# Autodesk Inventor assembly: ATP16XL025-A-P8
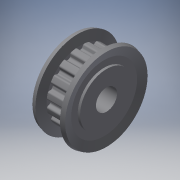
[picture p0: Inventor's stored thumbnail of the model, 180x180]
Saved by Autodesk Inventor 2019 (Build 230136000, 136)
## iProperties
Category: PARTsolutions
Company: MISUMI
Created: 2024-03-16
Part Number: ATP16XL025-A-P8
Catalog Web Link: www.cadenas.de
Description: ATP__XL025, ATP__XL031, ATP__ XL037, ATP__XL050, BTP__XL025, BTP__XL031, BTP__XL037, BTP__XL050, KTP__XL025, KTP__XL031, KTP__ XL037, KTP__XL050, NTP__XL025, NTP__XL031, NTP__ XL037, NTP__XL050, MTP__XL025, MTP__ XL037, MTP__XL050, MTPB__XL025, MTPB__ XL037, MTPB__XL050, MTPP__XL025, MTPP__ XL037, MTPP__XL050, STP__XL025, STP__XL031, STP__ XL037, STP__XL050, KATP__XL025, KATP__XL031, KATP__ XL037, KATP__XL050, KKTP__XL025, KKTP__XL031, KKTP__ XL037, KKTP__XL050-Timing Pulleys XL Type
Vendor: MISUMI
Document SubType Name: Assembly
Designer: psAdmin
Manufacturer: MISUMI
Mass: 5.87054 g
Surface Area: 39.0315 cm^2
Volume: 5.87054 cm^3
Density: 1 g/cm^3
Title: ATP16XL025-A-P8
Author: Cadenas PARTsolutions
Comments: Timing Pulleys XL Type
PSOL_IDENT_0: {$CADENAS_DATA/23d-libs/misumi/metric/51_timing_pulleys/mtp_xl_asmtab.prj},892 {VTYP=3D},{STYP=ASSTA
PSOL_IDENT_1: B},{NB=ATP16XL025-A-P8},{LINA=ATP16XL025-A-P8},{NN=ATP__XL025, ATP__XL031, ATP__ XL037, ATP__XL050,
PSOL_IDENT_2: BTP__XL025, BTP__XL031, BTP__XL037, BTP__XL050, KTP__XL025, KTP__XL031, KTP__ XL037, KTP__XL050, NTP
PSOL_IDENT_3: __XL025, NTP__XL031, NTP__ XL037, NTP__XL050, MTP__XL025, MTP__ XL037, MTP__XL050, MTPB__XL025, MTPB
PSOL_IDENT_4: __ XL037, MTPB__XL050, MTPP__XL025, MTPP__ XL037, MTPP__XL050, STP__XL025, STP__XL031, STP__ XL037,
PSOL_IDENT_5: STP__XL050, KATP__XL025, KATP__XL031, KATP__ XL037, KATP__XL050, KKTP__XL025, KKTP__XL031, KKTP__ XL
PSOL_IDENT_6: 037, KKTP__XL050},{DATE=06.01.2023 09:05:48},{GEOMDATE=06.01.2023 09:05:40},{VERSION=},{LINEID=30},{
PSOL_IDENT_7: WBVAR=MATP,ST,TNW,PS,SBS,DD,Z,J,Q,R,S,T,ALT1,ALT2,M,QSC,QFC,QTC,ALT3,K,KSC,KFC,KTC,ALT4,ZM,ZSC,ZFC,Z
PSOL_IDENT_8: TC,ALT5,ALT6,ALT7,FC,ALT8,SRG,ALT9,BTC,TL,ALT10,TPC,ALT11,BC,ALT12,SLH,ALT13,BN},{WBNUMERIC=DD,Z,J,Q
PSOL_IDENT_9: ,R,S,T,QSC,QFC,QTC,K,KSC,KFC,KTC,ZSC,ZFC,ZTC,FC,SRG,BTC,TL,BC,SLH,BN}  {NB=ATP16XL025-A-P8},{LINA=AT
PSOL_IDENT_10: P16XL025-A-P8},{KT=DUMMY},{PN=ATP16XL025-A-P8},{TYPE=ATP},{MATP=A2017},{MATPALG= 'A2017','Aluminum A
PSOL_IDENT_11: lloy 2000 series','S45C','1045 Carbon Steel Equivalent','SUS304','SUS304', 'A6000', '6000 Series Alu
PSOL_IDENT_12: minum Alloy' },{ST=CA},{STALG= 'CA','Clear Anodize','BA','Black Anodize','HAT','Hard Clear Anodize','
PSOL_IDENT_13: ENP','Electroless Nickel Plating' },{NT=16},{TNW=XL025},{TNWALG= 'XL025','XL031','XL037','XL050' },{
PSOL_IDENT_14: BW=6.4mm (1/4inch)},{PS=A},{PSALG= 'A','B' },{SBS=P},{SBSALG= 'H','Round Hole','P','Round Hole + Tap'
PSOL_IDENT_15: ,'N','New JIS Keywayed Bore + Tap (Standard)','NK','New JIS Keywayed Bore + Tap (width 4.0mm, height
PSOL_IDENT_16: 1.8mm)','C','Old JIS Keywayed Bore + Tap','V','Stepped Hole','Y','Both Ends Stepped Hole','WB','Dou
PSOL_IDENT_17: ble Stepped Hole' },{DD=8.00},{DDALG=[5:6/1],6.35,[7:12/1],12.7,[13:13/1]},{DDHA=[5:6/1],6.35,[7:12/
PSOL_IDENT_18: 1],12.7,[13:16/1]},{DDPA=[5:6/1],6.35,[7:12/1],12.7,[13:13/1]},{DDNA=[8:8/1],[10:13/1]},{DDNK=[10:10
PSOL_IDENT_19: /1]},{DDCA=[10,12]},{DDVA=[5:6/1],6.35,[7:12/1],12.7,[13:14/1]},{DDY=[5:14/1]},{DDWB=[5:12/1]},{DDHB=
PSOL_IDENT_20: },{DDPB=},{DDNB=},{DDCB=},{DDVFB=},{Z=0},{ZALG=[0]},{ZMIN=10.000},{ZAMAX=16.000},{ZBMAX=0.000},{DDZ=
PSOL_IDENT_21: 8.000},{J=0.0},{JALG=[0]},{JMIN=2.000},{JMAX=10.500},{JPN=},{Q=0},{QALG=[0]},{QRMIN=10.000},{QRMAX=1
PSOL_IDENT_22: 6},{WBQMIN=12.000},{R=0},{RALG=[0]},{WBRMAX=-2.000},{S=0.0},{SALG=[0]},{SMAX=6.5},{T=0.0},{TALG=[0]}
PSOL_IDENT_23: ,{TMAX=8},{SBSPN=-P8},{A=7.5},{W=12.5},{L=0},{PD=25.87},{OD=25.36},{D=0},{DALG=17.000},{DE=20},{F=32
PSOL_IDENT_24: },{E=20},{TT=1.6},{BBK=0.000},{TTK=0.0},{ALT1=},{ALT1ALG= '','w/o KC90 (Set Screw Angle)','KC90','wi
PSOL_IDENT_25: th KC90 (Set Screw Angle)' },{ANG=112.500},{ALT1PN=},{ALT2=},{ALT2ALG= '','Not applicable' },{M=N/A}
PSOL_IDENT_26: ,{MALG= 'N/A' },{MFTALG= 'N/A' },{MSALG= 'N/A' },{M3D=0.000},{KDML=0.000},{ML=0.000},{MUL=0.000},{PI
PSOL_IDENT_27: TCH=0.000},{QSC=0.0},{QSCALG=0},{QFC=0.0},{QFCALG=0},{QTC=0.0},{QTCALG=0},{QPCDMIN=0.000},{QPCDMINAL
PSOL_IDENT_28: G=0.000},{QPCDMAX=16.000},{ALT2PN=},{TAP=0.000},{ALT3=},{ALT3ALG= '','Not applicable' },{K=0.0},{KAL
PSOL_IDENT_29: G=0},{KMIN=4.000},{KFTMAX=0.000},{KSMAX=0.000},{KSC=0.0},{KSCALG=0},{KFC=0.0},{KFCALG=0},{KTC=0.0},{
PSOL_IDENT_30: KTCALG=0},{KSCMIN=12.000},{KPCDMIN=12.000},{KPCDMAX=16.000},{ALT3PN=},{ALT4=},{ALT4ALG= '','Not appl
PSOL_IDENT_31: icable' },{ALT4MIN=18.500},{ALT4MAX=9.500},{ZM=N/A},{ZMALG= 'N/A' },{ZMFTALG= 'N/A' },{ZMSALG= 'N/A'
PSOL_IDENT_32: },{ZMDD1=0.0},{ZMDD2=0.0},{ZMHH=0.0},{ZSC=0.0},{ZSCALG=[0]},{ZFC=0.0},{ZFCALG=[0]},{ZTC=0.0},{ZTCAL
PSOL_IDENT_33: G=[0]},{ZPCDMIN=0.000},{ZPCDMINALG=0.000},{ZPCDMAX=16.000},{ALT4PN=},{ALT5=},{ALT5ALG= '','w/o Flang
PSOL_IDENT_34: e not Attached','NFC','with NFC (Flange not Attached)' },{ALT5PN=},{ALT6=},{ALT6ALG= '','w/o Flange
PSOL_IDENT_35: Attached on One Side Only','RFC','with RFC (Flange Attached on The Boss Side Only)','LFC','with LFC
PSOL_IDENT_36: (Flange Attached on The Opposite Side Only)' },{ALT6PN=},{ALT7=},{ALT7ALG= '','w/o FC (Flange Cut)','
PSOL_IDENT_37: FC','with FC (Flange Cut)' },{FC=0.0},{FCALG=0},{FCMIN=26.5},{FCMAX=30.0},{ALT7PN=},{ALT8=},{ALT8ALG=
PSOL_IDENT_38: '','Not applicable' },{ALT8ALGALG=16.000},{ALT8DD2=0.000},{ALT8MM=0.000},{ALT8NN=0.000},{QC=0.000},
PSOL_IDENT_39: {KC=0.000},{ZC=0.000},{SRG=0.0},{SRGALG=[0]},{SRGMAX=0.000},{DD2=0.0},{MM=0.00},{NN=0.00},{ALT8PN=},
PSOL_IDENT_40: {ALT9=},{ALT9ALG= '','w/o BTC (Taper for Bearing Holder)','BTC','with BTC (Taper for Bearing Holder)'
PSOL_IDENT_41: },{BTC9=9.000},{TL9=1.000},{BTC=0},{BTCALG=[0]},{TL=0.0},{TLALG=0},{TLMIN=1.000},{TLMAX=-13.000},{B
PSOL_IDENT_42: TCL=0},{BTCD=0},{ALT9PN=},{WLBCTL=12.500},{ALT10=},{ALT10ALG= '','w/o TPC (Tapped Hole Dimension)','
PSOL_IDENT_43: TPC','with TPC (Tapped Hole Dimension)' },{TPC=N/A},{TPCALG= 'N/A' },{TPCM=4.000},{ALT10PN=},{ALT11=
PSOL_IDENT_44: },{ALT11ALG= '','Not applicable' },{BC=0.0},{BCALG=0},{BCMIN=7},{BCMAX=-13},{M1WBC=6.25},{ALT11PN=},
PSOL_IDENT_45: {KTT=8.68},{ALT12=},{ALT12ALG= '','w/o SLH (Set Screw Length)','SLH','with SLH (Set Screw Length)' }
PSOL_IDENT_46: ,{SLH=0},{SLHALG=[0]},{ALT12PN=},{ALT13=},{ALT13ALG= '', 'Not applicable' },{BN=0.0},{BNALG=0},{BNMI
PSOL_IDENT_47: N=-12},{BNMAX=-2.5},{ALT13PN=},{AC=M4x3},{M1=4.000},{M1L=3.000},{KEYA=1.000},{KEYB=0.000},{KEYM=1.00
PSOL_IDENT_48: 0},{PPATH=mtp_xl/mtp_xl_asmtpl.prj}
NB: ATP16XL025-A-P8
NN: 0
NT: 16
NBSYN: $PN.
LINA: ATP16XL025-A-P8
CATALOG: Misumi
PN: ATP16XL025-A-P8
MATP: Aluminum Alloy 2000 series
ST: Clear Anodize
TNW: XL025
BW: 6.4mm (1/4inch)
PS: A
SBS: Round Hole + Tap
DD: 8
Z: 0
J: 0
Q: 0
R: 0
S: 0
T: 0
A: 7.5
W: 12.5
L: 0
PD: 25.87
OD: 25.36
D: 0
F: 32
E: 20
TT: 1.6
ALT1: w/o KC90 (Set Screw Angle)
ALT2: Not applicable
M: N/A
QSC: 0
QFC: 0
QTC: 0
ALT3: Not applicable
K: 0
KSC: 0
KFC: 0
KTC: 0
ALT4: Not applicable
ZM: N/A
ZMDD1: 0
ZMDD2: 0
ZMHH: 0
ZSC: 0
ZFC: 0
ZTC: 0
ALT5: w/o Flange not Attached
ALT6: w/o Flange Attached on One Side Only
ALT7: w/o FC (Flange Cut)
FC: 0
ALT8: Not applicable
SRG: 0
DD2: 0
MM: 0
ALT9: w/o BTC (Taper for Bearing Holder)
BTC: 0
TL: 0
BTCL: 0
BTCD: 0
ALT10: w/o TPC (Tapped Hole Dimension)
TPC: N/A
ALT11: Not applicable
BC: 0
ALT12: w/o SLH (Set Screw Length)
SLH: 0
ALT13: Not applicable
BN: 0
AC: M4x3
SUPPLIER: MISUMI
ARTICLENO: ATP16XL025-A-P8
BOMINFO: ATP16XL025-A-P8
CREATOR: CADENAS GmbH
## Documents named in this file (3)
- e:\temp\worker_COMMON_2\temp\tmp_900_80_wLE1G\format_0\ATP16XL025-A-P8.iam
- e:\temp\worker_COMMON_2\temp\tmp_900_80_wLE1G\format_0\ATP16XL025-A-P8_b.ipt
- e:\temp\worker_COMMON_2\temp\tmp_900_80_wLE1G\format_0\SET-SCREW4-3.ipt
## Components (3 placed, 2 different names)
1. ATP16XL025-A-P8_b:1 — to_screw1_Z@1 <-> CP_Z@2, to_screw2_Z@1 <-> CP_Z@3
2. SET-SCREW4-3:1 — to_screw1_Z@1 <-> CP_Z@2
3. SET-SCREW4-3:2 — to_screw2_Z@1 <-> CP_Z@3
## Relationships (2: Mate 2)
- to_screw1_Z@1 <-> CP_Z@2 [Mate]: ATP16XL025-A-P8_b:1 ↔ SET-SCREW4-3:1
- to_screw2_Z@1 <-> CP_Z@3 [Mate]: ATP16XL025-A-P8_b:1 ↔ SET-SCREW4-3:2
